# Autodesk Inventor assembly: fourPmtDetector
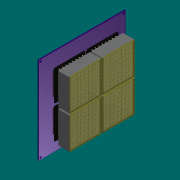
[picture p0: Inventor's stored thumbnail of the model, 180x180]
Saved by Autodesk Inventor 2016 (Build 200138000, 138)
## iProperties
Created: 2016-04-02
Part Number: fourPmtDetector
Document SubType Name: Assembly
Designer: sawai
Author: sawai
## Documents named in this file (3)
- C:\Users\sawaiz\oneDrive\projects\modularRICH\detector\fourPmtDetector.iam
- C:\Users\sawaiz\oneDrive\projects\modularRICH\detector\detectorArray.iam
- C:\Users\sawaiz\oneDrive\projects\modularRICH\dependency\modularRICHBackplane\cad\backplane.iam
## Components (3 placed, 2 different names)
1. detectorArray:1 [sub-assembly] — Flush:11, Mate:16, Mate:17, Angle:1, Flush:12
2. detectorArray:2 [sub-assembly] — Flush:11, Mate:16, Flush:12
3. backplane:1 [sub-assembly] — Mate:17, Angle:1
## Relationships (5: Flush 2, Mate 2, Angle 1)
- Flush:11: detectorArray:1 ↔ detectorArray:2
- Mate:16 (1 mm): detectorArray:1 ↔ detectorArray:2
- Mate:17: detectorArray:1 ↔ backplane:1
- Angle:1 (0 deg): detectorArray:1 ↔ backplane:1
- Flush:12: detectorArray:1 ↔ detectorArray:2
